# Autodesk Inventor assembly: Board Pattern
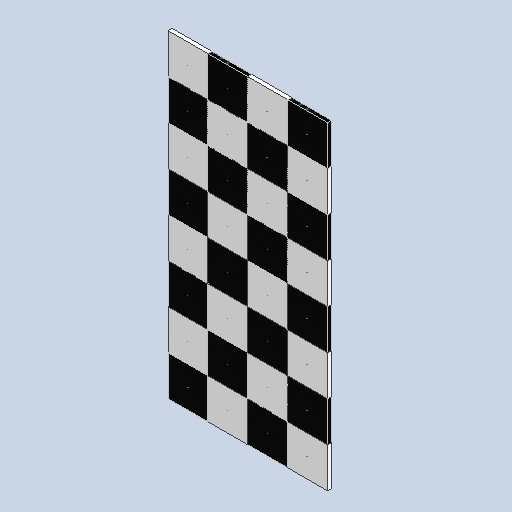
[picture p0: Inventor's stored thumbnail of the model, 512x512]
Saved by Autodesk Inventor 2022 (Build 260153000, 153)
## iProperties
Created: 2022-04-03
Part Number: Board Pattern
Document SubType Name: Assembly
Designer: Nick
Author: Nick
## Documents named in this file (3)
- Y:\Projects\Chess_Board\Board Pattern.iam
- Y:\Projects\Chess_Board\White Square.ipt
- Y:\Projects\Chess_Board\Black Square.ipt
## Components (32 placed, 2 different names)
1. White Square:1
2. Black Square:1
3. White Square:9
4. Black Square:9
5. White Square:10
6. Black Square:10
7. White Square:11
8. Black Square:11
9. White Square:12
10. Black Square:12
11. White Square:13
12. Black Square:13
13. White Square:14
14. Black Square:14
15. White Square:15
16. Black Square:15
17. White Square:16
18. Black Square:16
19. White Square:17
20. Black Square:17
21. White Square:18
22. Black Square:18
23. White Square:19
24. Black Square:19
25. White Square:20
26. Black Square:20
27. White Square:21
28. Black Square:21
29. White Square:22
30. Black Square:22
31. White Square:23
32. Black Square:23
## Component patterns: (8 elements, first: White Square:1 + Black Square:1 + White Square:9 + Black Square:9)
## Relationships (9: Flush 5, Mate 4)
- [Mate]: White Square:1 ↔ Black Square:1
- [Flush]: White Square:1 ↔ Black Square:1
- [Flush]: White Square:1 ↔ Black Square:1
- [Flush]: Black Square:1 ↔ White Square:9
- [Flush]: Black Square:1 ↔ White Square:9
- [Mate]: Black Square:1 ↔ White Square:9
- [Flush]: White Square:1 ↔ Black Square:9
- [Mate]: White Square:9 ↔ Black Square:9
- [Mate]: White Square:1 ↔ Black Square:9
## Named parameters: d16_d12 = 0 mm, d18_d14 = 0 mm
